# Autodesk Inventor assembly: Gripper
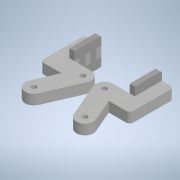
[picture p0: Inventor's stored thumbnail of the model, 180x180]
Saved by Autodesk Inventor 2020 (Build 240168000, 168)
## iProperties
Created: 2020-07-20
Part Number: Gripper
Document SubType Name: Assembly
Designer: WIN10
Author: WIN10
## Documents named in this file (5)
- C:\Users\WIN10\Downloads\Gripper.iam
- C:\Users\WIN10\Downloads\Chwytak wersja 3 - baza.ipt
- C:\Users\WIN10\Downloads\Chwytak wersja 3 - kwadrat.ipt
- C:\Users\WIN10\Downloads\Chwytak wersja 3 - baza_CPY.ipt
- C:\Users\WIN10\Downloads\Chwytak wersja 3 - kwadrat_CPY.ipt
## Components (4 placed, 4 different names)
1. Chwytak wersja 3 - baza:1 — Rigid:1
2. Chwytak wersja 3 - kwadrat:1 — Rigid:1
3. Chwytak wersja 3 - baza_CPY:1 — Rigid:2
4. Chwytak wersja 3 - kwadrat_CPY:1 — Rigid:2
## Relationships (2: WeldJoint 2)
- Rigid:1 [WeldJoint]: Chwytak wersja 3 - baza:1 ↔ Chwytak wersja 3 - kwadrat:1
- Rigid:2 [WeldJoint]: Chwytak wersja 3 - baza_CPY:1 ↔ Chwytak wersja 3 - kwadrat_CPY:1
